# Autodesk Inventor assembly: Montagem traseiro
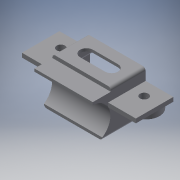
[picture p0: Inventor's stored thumbnail of the model, 180x180]
Saved by Autodesk Inventor 2019 (Build 230136000, 136)
## iProperties
Created: 2021-06-28
Part Number: Montagem traseiro
Material: Genérico
Document SubType Name: Assembly
Designer: SOU O MELHOR
Author: SOU O MELHOR
## Documents named in this file (3)
- F:\Lucas\BAJA\Inventor\Atividades\Nova fixação do acelerometro 2\Montagem traseiro.iam
- F:\Lucas\BAJA\Inventor\Atividades\Nova fixação do acelerometro 2\Caixa traseira.ipt
- F:\Lucas\BAJA\Inventor\Atividades\Nova fixação do acelerometro 2\Fixador traseiro.ipt
## Components (2 placed, 2 different names)
1. Caixa traseira:1 — Coincidência:1, Coincidência:2
2. Fixador traseiro:1 — Coincidência:1, Coincidência:2
## Relationships (2: Mate 2)
- Coincidência:1 [Mate]: Caixa traseira:1 ↔ Fixador traseiro:1
- Coincidência:2 [Mate]: Caixa traseira:1 ↔ Fixador traseiro:1
